# Autodesk Inventor assembly: Superstructure-Mount
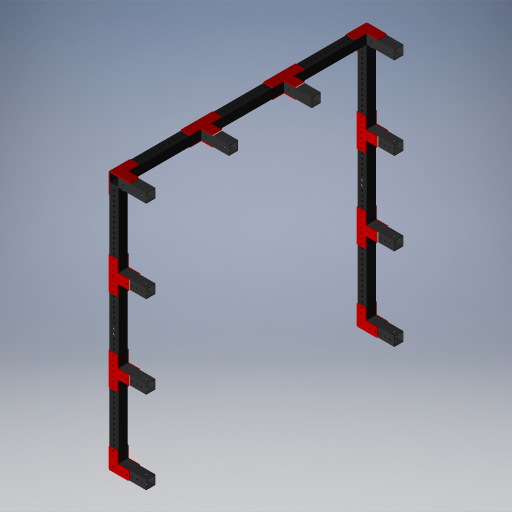
[picture p0: Inventor's stored thumbnail of the model, 512x512]
Saved by Autodesk Inventor 2024.2 (Build 282272000, 272)
## iProperties
Created: 2024-02-11
Part Number: Superstructure-Mount
Document SubType Name: Assembly
Designer: rohan
Author: rohan
## Documents named in this file (6)
- C:\Users\rohan\OneDrive - Hillsborough County Public Schools\Robotics\FIRST-Robotics-Competition\Crescendo\Minotaur-Crescendo-Robot\Structure\Aluminum-Extrusions\Superstructure-Mount.iam
- C:\Users\rohan\OneDrive - Hillsborough County Public Schools\Robotics\FIRST-Robotics-Competition\Crescendo\Minotaur-Crescendo-Robot\Structure\Aluminum-Extrusions\2024-100-009-Structure-Front-Rail.ipt
- C:\Users\rohan\OneDrive - Hillsborough County Public Schools\Robotics\FIRST-Robotics-Competition\Crescendo\Minotaur-Crescendo-Robot\Structure\Aluminum-Extrusions\2024-100-008-Structure-Standoffs.ipt
- C:\Users\rohan\OneDrive - Hillsborough County Public Schools\Robotics\FIRST-Robotics-Competition\Crescendo\Minotaur-Crescendo-Robot\Structure\Aluminum-Extrusions\2024-100-009-Structure-Side-Rail.ipt
- C:\Users\rohan\OneDrive - Hillsborough County Public Schools\Robotics\FIRST-Robotics-Competition\Crescendo\Minotaur-Crescendo-Robot\Structure\Gussets\Custom-Superstructure-Mount-T-Gusset.ipt
- C:\Users\rohan\OneDrive - Hillsborough County Public Schools\Robotics\FIRST-Robotics-Competition\Crescendo\Minotaur-Crescendo-Robot\Structure\Gussets\Custom-Superstructure-Mount-L-Gusset.ipt
## Components (33 placed, 5 different names)
1. 2024-100-009-Structure-Front-Rail:1 — Mate:1, Flush:1, Flush:2, Mate:2, Flush:3, Flush:4, Mate:3, Mate:4, Flush:5, Flush:6, Mate:7, Flush:7, Flush:8, Mate:8, Flush:9, Flush:10, Mate:32, Flush:45, Mate:33, Flush:47, Mate:40, Flush:62, Mate:41, Flush:63, Mate:42, Flush:65, Mate:43, Flush:67
2. 2024-100-008-Structure-Standoffs:1 — Mate:2, Flush:3, Flush:4, Mate:5, Mate:17, Flush:68
3. 2024-100-008-Structure-Standoffs:2 — Mate:1, Flush:1, Flush:2, Mate:6, Flush:15, Mate:14, Flush:66
4. 2024-100-008-Structure-Standoffs:3 — Mate:3, Flush:5, Mate:5, Flush:48
5. 2024-100-008-Structure-Standoffs:4 — Mate:4, Flush:6, Mate:6, Flush:46
6. 2024-100-009-Structure-Side-Rail:1 — Mate:7, Flush:7, Flush:8, Mate:10, Flush:13, Flush:14, Mate:11, Mate:12, Flush:31, Mate:25, Flush:35, Mate:27, Flush:58, Mate:38, Flush:64
7. 2024-100-009-Structure-Side-Rail:2 — Mate:8, Flush:9, Flush:10, Mate:9, Flush:11, Flush:12, Mate:15, Mate:16, Flush:17, Flush:18, Mate:34, Flush:49, Flush:51, Mate:35, Mate:39, Flush:59, Flush:61
8. 2024-100-008-Structure-Standoffs:5 — Mate:10, Flush:13, Flush:14, Flush:16, Mate:13, Flush:57
9. 2024-100-008-Structure-Standoffs:6 — Mate:9, Flush:11, Flush:12, Mate:18, Flush:60
10. 2024-100-008-Structure-Standoffs:7 — Mate:12, Flush:15, Mate:14, Flush:36
11. 2024-100-008-Structure-Standoffs:8 — Mate:11, Flush:16, Mate:13, Flush:32
12. 2024-100-008-Structure-Standoffs:9 — Mate:16, Flush:18, Mate:17, Flush:50
13. 2024-100-008-Structure-Standoffs:10 — Mate:15, Flush:17, Mate:18, Flush:52
14. Custom-Superstructure-Mount-T-Gusset:1 — Flush:19, Flush:20, Mate:19, Flush:31, Flush:32
15. Custom-Superstructure-Mount-T-Gusset:2 — Flush:19, Flush:20, Mate:19, Mate:25
16. Custom-Superstructure-Mount-T-Gusset:13 — Flush:35, Flush:36, Mate:27
17. Custom-Superstructure-Mount-T-Gusset:14
18. Custom-Superstructure-Mount-T-Gusset:15
19. Custom-Superstructure-Mount-T-Gusset:16 — Mate:32, Flush:45, Flush:46
20. Custom-Superstructure-Mount-T-Gusset:17
21. Custom-Superstructure-Mount-T-Gusset:18 — Mate:33, Flush:47, Flush:48
22. Custom-Superstructure-Mount-T-Gusset:19
23. Custom-Superstructure-Mount-T-Gusset:20 — Mate:34, Flush:49, Flush:50
24. Custom-Superstructure-Mount-T-Gusset:21 — Flush:51, Flush:52
25. Custom-Superstructure-Mount-T-Gusset:22 — Mate:35
26. Custom-Superstructure-Mount-L-Gusset:1 — Flush:53, Flush:54, Mate:36, Mate:38
27. Custom-Superstructure-Mount-L-Gusset:2 — Flush:53, Flush:54, Mate:36, Flush:57, Flush:58
28. Custom-Superstructure-Mount-L-Gusset:3 — Flush:59, Flush:60
29. Custom-Superstructure-Mount-L-Gusset:4 — Mate:39
30. Custom-Superstructure-Mount-L-Gusset:5 — Mate:41, Flush:63, Flush:64
31. Custom-Superstructure-Mount-L-Gusset:6 — Mate:40, Flush:61, Flush:62
32. Custom-Superstructure-Mount-L-Gusset:7 — Mate:42, Flush:65, Flush:66
33. Custom-Superstructure-Mount-L-Gusset:8 — Mate:43, Flush:67, Flush:68
## Relationships (96: Flush 58, Mate 38)
- Mate:1: 2024-100-009-Structure-Front-Rail:1 ↔ 2024-100-008-Structure-Standoffs:2
- Flush:1: 2024-100-009-Structure-Front-Rail:1 ↔ 2024-100-008-Structure-Standoffs:2
- Flush:2: 2024-100-009-Structure-Front-Rail:1 ↔ 2024-100-008-Structure-Standoffs:2
- Mate:2: 2024-100-009-Structure-Front-Rail:1 ↔ 2024-100-008-Structure-Standoffs:1
- Flush:3: 2024-100-009-Structure-Front-Rail:1 ↔ 2024-100-008-Structure-Standoffs:1
- Flush:4: 2024-100-009-Structure-Front-Rail:1 ↔ 2024-100-008-Structure-Standoffs:1
- Mate:3: 2024-100-009-Structure-Front-Rail:1 ↔ 2024-100-008-Structure-Standoffs:3
- Mate:4: 2024-100-009-Structure-Front-Rail:1 ↔ 2024-100-008-Structure-Standoffs:4
- Flush:5: 2024-100-009-Structure-Front-Rail:1 ↔ 2024-100-008-Structure-Standoffs:3
- Flush:6: 2024-100-009-Structure-Front-Rail:1 ↔ 2024-100-008-Structure-Standoffs:4
- Mate:5 (203.2 mm): 2024-100-008-Structure-Standoffs:1 ↔ 2024-100-008-Structure-Standoffs:3
- Mate:6 (203.2 mm): 2024-100-008-Structure-Standoffs:2 ↔ 2024-100-008-Structure-Standoffs:4
- Mate:7: 2024-100-009-Structure-Front-Rail:1 ↔ 2024-100-009-Structure-Side-Rail:1
- Flush:7: 2024-100-009-Structure-Front-Rail:1 ↔ 2024-100-009-Structure-Side-Rail:1
- Flush:8: 2024-100-009-Structure-Front-Rail:1 ↔ 2024-100-009-Structure-Side-Rail:1
- Mate:8: 2024-100-009-Structure-Front-Rail:1 ↔ 2024-100-009-Structure-Side-Rail:2
- Flush:9: 2024-100-009-Structure-Front-Rail:1 ↔ 2024-100-009-Structure-Side-Rail:2
- Flush:10: 2024-100-009-Structure-Front-Rail:1 ↔ 2024-100-009-Structure-Side-Rail:2
- Mate:9: 2024-100-009-Structure-Side-Rail:2 ↔ 2024-100-008-Structure-Standoffs:6
- Flush:11: 2024-100-009-Structure-Side-Rail:2 ↔ 2024-100-008-Structure-Standoffs:6
- Flush:12: 2024-100-009-Structure-Side-Rail:2 ↔ 2024-100-008-Structure-Standoffs:6
- Mate:10: 2024-100-009-Structure-Side-Rail:1 ↔ 2024-100-008-Structure-Standoffs:5
- Flush:13: 2024-100-009-Structure-Side-Rail:1 ↔ 2024-100-008-Structure-Standoffs:5
- Flush:14: 2024-100-009-Structure-Side-Rail:1 ↔ 2024-100-008-Structure-Standoffs:5
- Mate:11: 2024-100-009-Structure-Side-Rail:1 ↔ 2024-100-008-Structure-Standoffs:8
- Mate:12: 2024-100-009-Structure-Side-Rail:1 ↔ 2024-100-008-Structure-Standoffs:7
- Flush:15: 2024-100-008-Structure-Standoffs:2 ↔ 2024-100-008-Structure-Standoffs:7
- Flush:16: 2024-100-008-Structure-Standoffs:5 ↔ 2024-100-008-Structure-Standoffs:8
- Mate:13 (203.2 mm): 2024-100-008-Structure-Standoffs:5 ↔ 2024-100-008-Structure-Standoffs:8
- Mate:14 (203.2 mm): 2024-100-008-Structure-Standoffs:2 ↔ 2024-100-008-Structure-Standoffs:7
- Mate:15: 2024-100-009-Structure-Side-Rail:2 ↔ 2024-100-008-Structure-Standoffs:10
- Mate:16: 2024-100-009-Structure-Side-Rail:2 ↔ 2024-100-008-Structure-Standoffs:9
- Flush:17: 2024-100-009-Structure-Side-Rail:2 ↔ 2024-100-008-Structure-Standoffs:10
- Flush:18: 2024-100-009-Structure-Side-Rail:2 ↔ 2024-100-008-Structure-Standoffs:9
- Mate:17 (203.2 mm): 2024-100-008-Structure-Standoffs:1 ↔ 2024-100-008-Structure-Standoffs:9
- Mate:18 (203.2 mm): 2024-100-008-Structure-Standoffs:6 ↔ 2024-100-008-Structure-Standoffs:10
- Flush:19: Custom-Superstructure-Mount-T-Gusset:1 ↔ Custom-Superstructure-Mount-T-Gusset:2
- Flush:20: Custom-Superstructure-Mount-T-Gusset:1 ↔ Custom-Superstructure-Mount-T-Gusset:2
- Mate:19 (25.4 mm): Custom-Superstructure-Mount-T-Gusset:1 ↔ Custom-Superstructure-Mount-T-Gusset:2
- Flush:31: 2024-100-009-Structure-Side-Rail:1 ↔ Custom-Superstructure-Mount-T-Gusset:1
- Mate:25: 2024-100-009-Structure-Side-Rail:1 ↔ Custom-Superstructure-Mount-T-Gusset:2
- Flush:32: 2024-100-008-Structure-Standoffs:8 ↔ Custom-Superstructure-Mount-T-Gusset:1
- [Flush]: Custom-Superstructure-Mount-T-Gusset:13 ↔ Custom-Superstructure-Mount-T-Gusset:14
- [Flush]: Custom-Superstructure-Mount-T-Gusset:13 ↔ Custom-Superstructure-Mount-T-Gusset:14
- [Mate] (25.4 mm): Custom-Superstructure-Mount-T-Gusset:13 ↔ Custom-Superstructure-Mount-T-Gusset:14
- Flush:35: 2024-100-009-Structure-Side-Rail:1 ↔ Custom-Superstructure-Mount-T-Gusset:13
- Flush:36: 2024-100-008-Structure-Standoffs:7 ↔ Custom-Superstructure-Mount-T-Gusset:13
- Mate:27: 2024-100-009-Structure-Side-Rail:1 ↔ Custom-Superstructure-Mount-T-Gusset:13
- [Flush]: Custom-Superstructure-Mount-T-Gusset:15 ↔ Custom-Superstructure-Mount-T-Gusset:16
- [Flush]: Custom-Superstructure-Mount-T-Gusset:15 ↔ Custom-Superstructure-Mount-T-Gusset:16
- [Mate] (25.4 mm): Custom-Superstructure-Mount-T-Gusset:15 ↔ Custom-Superstructure-Mount-T-Gusset:16
- [Flush]: Custom-Superstructure-Mount-T-Gusset:17 ↔ Custom-Superstructure-Mount-T-Gusset:18
- [Flush]: Custom-Superstructure-Mount-T-Gusset:17 ↔ Custom-Superstructure-Mount-T-Gusset:18
- [Mate] (25.4 mm): Custom-Superstructure-Mount-T-Gusset:17 ↔ Custom-Superstructure-Mount-T-Gusset:18
- [Flush]: Custom-Superstructure-Mount-T-Gusset:19 ↔ Custom-Superstructure-Mount-T-Gusset:20
- [Flush]: Custom-Superstructure-Mount-T-Gusset:19 ↔ Custom-Superstructure-Mount-T-Gusset:20
- [Mate] (25.4 mm): Custom-Superstructure-Mount-T-Gusset:19 ↔ Custom-Superstructure-Mount-T-Gusset:20
- [Flush]: Custom-Superstructure-Mount-T-Gusset:21 ↔ Custom-Superstructure-Mount-T-Gusset:22
- [Flush]: Custom-Superstructure-Mount-T-Gusset:21 ↔ Custom-Superstructure-Mount-T-Gusset:22
- [Mate] (25.4 mm): Custom-Superstructure-Mount-T-Gusset:21 ↔ Custom-Superstructure-Mount-T-Gusset:22
- Mate:32: 2024-100-009-Structure-Front-Rail:1 ↔ Custom-Superstructure-Mount-T-Gusset:16
- Flush:45: 2024-100-009-Structure-Front-Rail:1 ↔ Custom-Superstructure-Mount-T-Gusset:16
- Flush:46: 2024-100-008-Structure-Standoffs:4 ↔ Custom-Superstructure-Mount-T-Gusset:16
- Mate:33: 2024-100-009-Structure-Front-Rail:1 ↔ Custom-Superstructure-Mount-T-Gusset:18
- Flush:47: 2024-100-009-Structure-Front-Rail:1 ↔ Custom-Superstructure-Mount-T-Gusset:18
- Flush:48: 2024-100-008-Structure-Standoffs:3 ↔ Custom-Superstructure-Mount-T-Gusset:18
- Mate:34: 2024-100-009-Structure-Side-Rail:2 ↔ Custom-Superstructure-Mount-T-Gusset:20
- Flush:49: 2024-100-009-Structure-Side-Rail:2 ↔ Custom-Superstructure-Mount-T-Gusset:20
- Flush:50: 2024-100-008-Structure-Standoffs:9 ↔ Custom-Superstructure-Mount-T-Gusset:20
- Flush:51: 2024-100-009-Structure-Side-Rail:2 ↔ Custom-Superstructure-Mount-T-Gusset:21
- Mate:35: 2024-100-009-Structure-Side-Rail:2 ↔ Custom-Superstructure-Mount-T-Gusset:22
- Flush:52: 2024-100-008-Structure-Standoffs:10 ↔ Custom-Superstructure-Mount-T-Gusset:21
- Flush:53: Custom-Superstructure-Mount-L-Gusset:1 ↔ Custom-Superstructure-Mount-L-Gusset:2
- Flush:54: Custom-Superstructure-Mount-L-Gusset:1 ↔ Custom-Superstructure-Mount-L-Gusset:2
- Mate:36 (25.4 mm): Custom-Superstructure-Mount-L-Gusset:1 ↔ Custom-Superstructure-Mount-L-Gusset:2
- [Flush]: Custom-Superstructure-Mount-L-Gusset:3 ↔ Custom-Superstructure-Mount-L-Gusset:4
- [Flush]: Custom-Superstructure-Mount-L-Gusset:3 ↔ Custom-Superstructure-Mount-L-Gusset:4
- [Mate] (25.4 mm): Custom-Superstructure-Mount-L-Gusset:3 ↔ Custom-Superstructure-Mount-L-Gusset:4
- Flush:57: 2024-100-008-Structure-Standoffs:5 ↔ Custom-Superstructure-Mount-L-Gusset:2
- Flush:58: 2024-100-009-Structure-Side-Rail:1 ↔ Custom-Superstructure-Mount-L-Gusset:2
- Mate:38: 2024-100-009-Structure-Side-Rail:1 ↔ Custom-Superstructure-Mount-L-Gusset:1
- Mate:39: 2024-100-009-Structure-Side-Rail:2 ↔ Custom-Superstructure-Mount-L-Gusset:4
- Flush:59: 2024-100-009-Structure-Side-Rail:2 ↔ Custom-Superstructure-Mount-L-Gusset:3
- Flush:60: 2024-100-008-Structure-Standoffs:6 ↔ Custom-Superstructure-Mount-L-Gusset:3
- Mate:40: 2024-100-009-Structure-Front-Rail:1 ↔ Custom-Superstructure-Mount-L-Gusset:6
- Flush:61: 2024-100-009-Structure-Side-Rail:2 ↔ Custom-Superstructure-Mount-L-Gusset:6
- Flush:62: 2024-100-009-Structure-Front-Rail:1 ↔ Custom-Superstructure-Mount-L-Gusset:6
- Mate:41: 2024-100-009-Structure-Front-Rail:1 ↔ Custom-Superstructure-Mount-L-Gusset:5
- Flush:63: 2024-100-009-Structure-Front-Rail:1 ↔ Custom-Superstructure-Mount-L-Gusset:5
- Flush:64: 2024-100-009-Structure-Side-Rail:1 ↔ Custom-Superstructure-Mount-L-Gusset:5
- Mate:42: 2024-100-009-Structure-Front-Rail:1 ↔ Custom-Superstructure-Mount-L-Gusset:7
- Flush:65: 2024-100-009-Structure-Front-Rail:1 ↔ Custom-Superstructure-Mount-L-Gusset:7
- Flush:66: 2024-100-008-Structure-Standoffs:2 ↔ Custom-Superstructure-Mount-L-Gusset:7
- Mate:43: 2024-100-009-Structure-Front-Rail:1 ↔ Custom-Superstructure-Mount-L-Gusset:8
- Flush:67: 2024-100-009-Structure-Front-Rail:1 ↔ Custom-Superstructure-Mount-L-Gusset:8
- Flush:68: 2024-100-008-Structure-Standoffs:1 ↔ Custom-Superstructure-Mount-L-Gusset:8
## Named parameters: d57_d36 = 0 mm, d58_d37 = 0 mm, d59_d38 = 25.4 mm, d63_d57_d36 = 0 mm, d64_d58_d37 = 0 mm, d65_d59_d38 = 25.4 mm, d66_d57_d36 = 0 mm, d67_d58_d37 = 0 mm, d68_d59_d38 = 25.4 mm, d69_d57_d36 = 0 mm, d70_d58_d37 = 0 mm, d71_d59_d38 = 25.4 mm, d72_d57_d36 = 0 mm, d73_d58_d37 = 0 mm, d74_d59_d38 = 25.4 mm, d90_d87 = 0 mm, d91_d88 = 0 mm, d92_d89 = 25.4 mm
